# Autodesk Inventor assembly: FR-06assembled
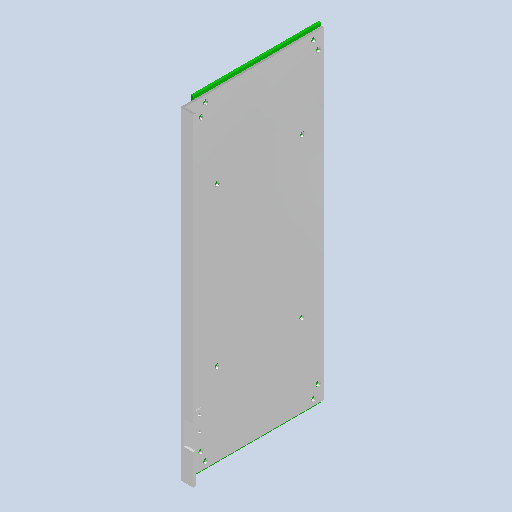
[picture p0: Inventor's stored thumbnail of the model, 512x512]
Saved by Autodesk Inventor 2022 (Build 260153000, 153)
## iProperties
Created: 2021-10-08
Part Number: FR-06assembled
Document SubType Name: Assembly
Designer: Bowen O'Steen
Author: Bowen O'Steen
## Documents named in this file (3)
- C:\$WorkingFolder\Engineering Data\MemeSat\Assembly\FR-06assembled.iam
- C:\$WorkingFolder\Engineering Data\MemeSat\Frame\FR-Default.ipt
- C:\$WorkingFolder\Engineering Data\MemeSat\Solar Panels\SP.iam
## Components (2 placed, 2 different names)
1. FR-Default:1 — Mate:1, Mate:2, Flush:1, Mate:3, Mate:4, Mate:5
2. SP:1 [sub-assembly] — Mate:3, Mate:4, Mate:5
## Relationships (6: Mate 5, Flush 1)
- Mate:1: FR-Default:1
- Mate:2: FR-Default:1
- Flush:1: FR-Default:1
- Mate:3: FR-Default:1 ↔ SP:1
- Mate:4: FR-Default:1 ↔ SP:1
- Mate:5: FR-Default:1 ↔ SP:1
